# Autodesk Inventor assembly: BV-ASM-222-102
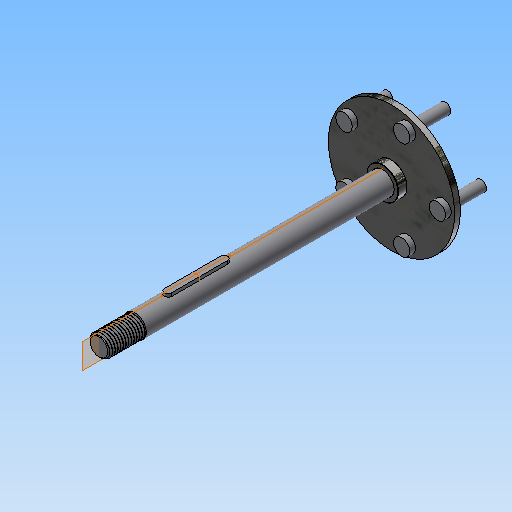
[picture p0: Inventor's stored thumbnail of the model, 512x512]
Saved by Autodesk Inventor 2025.4 (Build 294407000, 407)
## iProperties
RuleStatus: InUse
Created: 2022-04-22
Part Number: BV-ASM-222-102
Document SubType Name: Assembly
Designer: josh Hofer
Description: WHEEL SHAFT ASSEMBLY
Mass: 905.145 g
Surface Area: 752.944 cm^2
Volume: 284.369 cm^3
Density: 3.183 g/cm^3
Author: josh Hofer
Revision Number: ANY
## iProperties of the stored document MemberDocs/xJbdrnimgPssx2lthSyk151gfPd
RuleStatus: InUse
Created: 2022-04-22
Part Number: BV-ASM-222-102
Document SubType Name: Assembly
Designer: josh Hofer
Description: WHEEL SHAFT ASSEMBLY
Mass: 905.145 g
Surface Area: 752.944 cm^2
Volume: 284.369 cm^3
Density: 3.183 g/cm^3
Author: josh Hofer
Revision Number: ANY
## Documents named in this file (6)
- R:\A1- Neuweg Design Data\OM Robotics\BASE VEHICLE DESIGN PROJECT\BV-ASM-222-102.iam
- R:\A1- Neuweg Design Data\OM Robotics\BASE VEHICLE DESIGN PROJECT\0222-113.ipt
- R:\A1- Neuweg Design Data\OM Robotics\BASE VEHICLE DESIGN PROJECT\0222-108.ipt
- R:\A1- Neuweg Design Data\OM Robotics\BASE VEHICLE DESIGN PROJECT\0222-107.ipt
- R:\A1- Neuweg Design Data\OM Robotics\BASE VEHICLE DESIGN PROJECT\96717A416.ipt
- R:\A1- Neuweg Design Data\OM Robotics\BASE VEHICLE DESIGN PROJECT\M12-1.50.ipt
## Components (9 placed, 9 different names)
1. 0222-107 wheel shaft_344 — Insert:1, Mate:1, Mate:2, Mate:3, Flush:1, Flush:2
2. 0222-108 wheel hub adapter_345 — Insert:1, Insert:2, Insert:3, Insert:4, Insert:5, Insert:6, Insert:7, Mate:1, Insert:15
3. M12-1.50 wheel stud_346 — Insert:4
4. M12-1.50 wheel stud_347 — Insert:3
5. M12-1.50 wheel stud_348 — Insert:6
6. M12-1.50 wheel stud_349 — Insert:5
7. M12-1.50 wheel stud_350 — Insert:2, Insert:7
8. 0222-113:1 — Insert:15
9. 96717A416:1 — Mate:2, Mate:3, Flush:1
## Relationships (13: Insert 8, Mate 3, Flush 2)
- Insert:1 (12.7 mm): 0222-107 wheel shaft_344 ↔ 0222-108 wheel hub adapter_345
- Insert:2: 0222-108 wheel hub adapter_345 ↔ M12-1.50 wheel stud_350
- Insert:3: 0222-108 wheel hub adapter_345 ↔ M12-1.50 wheel stud_347
- Insert:4: 0222-108 wheel hub adapter_345 ↔ M12-1.50 wheel stud_346
- Insert:5: 0222-108 wheel hub adapter_345 ↔ M12-1.50 wheel stud_349
- Insert:6: 0222-108 wheel hub adapter_345 ↔ M12-1.50 wheel stud_348
- Insert:7: 0222-108 wheel hub adapter_345 ↔ M12-1.50 wheel stud_350
- Mate:1: 0222-107 wheel shaft_344 ↔ 0222-108 wheel hub adapter_345
- Insert:15: 0222-108 wheel hub adapter_345 ↔ 0222-113:1
- Mate:2: 0222-107 wheel shaft_344 ↔ 96717A416:1
- Mate:3: 0222-107 wheel shaft_344 ↔ 96717A416:1
- Flush:1 (-107.569 mm): 0222-107 wheel shaft_344 ↔ 96717A416:1
- Flush:2 (-107.5512 mm): 0222-107 wheel shaft_344
